# Autodesk Inventor assembly: painel
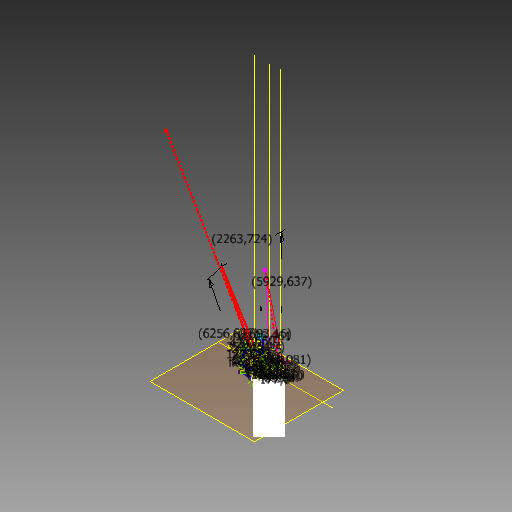
[picture p0: Inventor's stored thumbnail of the model, 512x512]
Saved by Autodesk Inventor 2019 (Build 230136000, 136)
## iProperties
Created: 2020-05-31
Part Number: painel
Document SubType Name: Assembly
Designer: luiza
Author: luiza
## Documents named in this file (8)
- G:\Meu Drive\Projetos\Projeto 2020 2021\Eletrônica 2020-2021\Projeção mecânica\Painel\painel.iam
- G:\Meu Drive\Projetos\Projeto 2020 2021\Eletrônica 2020-2021\Projeção mecânica\Painel\Caixa Painel.ipt
- G:\Meu Drive\Projetos\Projeto 2020 2021\Eletrônica 2020-2021\Projeção mecânica\Painel\Espaçadores.ipt
- G:\Meu Drive\Projetos\Projeto 2020 2021\Eletrônica 2020-2021\Projeção mecânica\Painel\Fixação Painel.ipt
- G:\Meu Drive\Projetos\Projeto 2020 2021\Eletrônica 2020-2021\Projeção mecânica\Painel\Tampa Painel.ipt
- G:\Meu Drive\Projetos\Projeto 2020 2021\Eletrônica 2020-2021\Projeção mecânica\Painel\LCD12864_st7920.iam
- G:\Meu Drive\Projetos\Projeto 2020 2021\Suspensão & Direção 2020_2021\Geometrias\Geometria Suspensão e Direção.iam
- G:\Meu Drive\Projetos\Projeto 2020 2021\Eletrônica 2020-2021\Projeção mecânica\Painel\painel\Frame\Frame0001.iam
## Components (11 placed, 7 different names)
1. Tampa Painel:1 — Flush:1, Mate:1, Mate:2, Mate:3, Mate:4, Mate:5, Mate:6, Flush:2, Flush:3, Mate:11, Mate:13, Mate:14, Angle:1
2. LCD12864_st7920:1 [sub-assembly] — Flush:1, Mate:1, Mate:2, Mate:7, Mate:8, Mate:9, Mate:10
3. Caixa Painel:1 — Flush:2, Flush:3, Mate:11, Mate:15, Mate:16, Flush:9
4. Espaçadores:1 — Mate:3, Mate:8
5. Espaçadores:2 — Mate:4, Mate:9
6. Espaçadores:3 — Mate:5, Mate:10
7. Espaçadores:4 — Mate:6, Mate:7
8. Fixação Painel:1 — Mate:12, Flush:4, Flush:5, Mate:14, Mate:15, Mate:16
9. Fixação Painel:2 — Mate:12, Flush:4, Flush:5, Mate:13, Mate:17
10. Geometria Suspensão e Direção:1 [sub-assembly] — Flush:6, Flush:7, Flush:8
11. Frame0001:1 [sub-assembly] — Mate:17
## Relationships (28: Mate 17, Flush 10, Angle 1)
- Flush:1: Tampa Painel:1 ↔ LCD12864_st7920:1
- Mate:1 (0.2 mm): Tampa Painel:1 ↔ LCD12864_st7920:1
- Mate:2 (0.2 mm): Tampa Painel:1 ↔ LCD12864_st7920:1
- Mate:3: Tampa Painel:1 ↔ Espaçadores:1
- Mate:4: Tampa Painel:1 ↔ Espaçadores:2
- Mate:5: Tampa Painel:1 ↔ Espaçadores:3
- Mate:6: Tampa Painel:1 ↔ Espaçadores:4
- Mate:7: LCD12864_st7920:1 ↔ Espaçadores:4
- Mate:8: LCD12864_st7920:1 ↔ Espaçadores:1
- Mate:9: LCD12864_st7920:1 ↔ Espaçadores:2
- Mate:10: LCD12864_st7920:1 ↔ Espaçadores:3
- Flush:2: Tampa Painel:1 ↔ Caixa Painel:1
- Flush:3: Tampa Painel:1 ↔ Caixa Painel:1
- Mate:11: Tampa Painel:1 ↔ Caixa Painel:1
- Mate:12 (150 mm): Fixação Painel:1 ↔ Fixação Painel:2
- Flush:4: Fixação Painel:1 ↔ Fixação Painel:2
- Flush:5: Fixação Painel:1 ↔ Fixação Painel:2
- Mate:13: Tampa Painel:1 ↔ Fixação Painel:2
- Mate:14 (-35 mm): Tampa Painel:1 ↔ Fixação Painel:1
- Mate:15: Caixa Painel:1 ↔ Fixação Painel:1
- Mate:16: Caixa Painel:1 ↔ Fixação Painel:1
- Flush:6: Geometria Suspensão e Direção:1
- Flush:7: Geometria Suspensão e Direção:1
- Flush:8: Geometria Suspensão e Direção:1
- Flush:9 (-75 mm): Caixa Painel:1
- Flush:10 (75 mm)
- Angle:1 (45 deg): Tampa Painel:1
- Mate:17: Fixação Painel:2 ↔ Frame0001:1
